# Autodesk Inventor assembly: MG996R_Servo_Motor_WithHorn
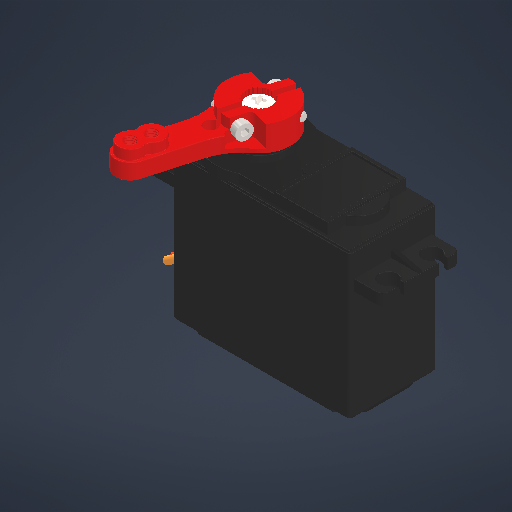
[picture p0: Inventor's stored thumbnail of the model, 512x512]
Saved by Autodesk Inventor 2025.2 (Build 292293000, 293)
## iProperties
Created: 2023-11-19
Part Number: MG996R_Servo_Motor_WithHorn
Document SubType Name: Assembly
Designer: Tiago
Sending System: SolidWorks 2022
Last Author: Ayman
Last Saved: 2023-12-26
Author: Tiago
## Documents named in this file (7)
- C:\Users\Tiago\Documents\Inventor\Exp. Braço v1\MG996R_Servo_Motor_WithHorn.iam
- C:\Users\Tiago\Documents\Inventor\Exp. Braço v1\MG996R Servo Motor\MG996R Servo Motor\MG996R Servo Motor\Case.ipt
- C:\Users\Tiago\Documents\Inventor\Exp. Braço v1\MG996R Servo Motor\MG996R Servo Motor\MG996R Servo Motor\Output Shaft.ipt
- C:\Users\Tiago\Documents\Inventor\Exp. Braço v1\MG996R Servo Motor\MG996R Servo Motor\MG996R Servo Motor\Rubber Wire Cable Sleeve.ipt
- C:\Users\Tiago\Documents\Inventor\Exp. Braço v1\MG996R Servo Motor\MG996R Servo Motor\MG996R Servo Motor\Pan Head Cross Screw M1.6.ipt
- C:\Users\Tiago\Documents\Inventor\Exp. Braço v1\MG996R Servo Motor\MG996R Servo Motor\MG996R Servo Motor\Pan Head Cross Screw M3.ipt
- C:\Users\Tiago\Documents\Inventor\Exp. Braço v1\SERVO ARM HORN 25T ALUMINIUM\SERVO ARM HORN WITH FASTENERS\SERVO ARM HORN WITH FASTENERS\SERVO ARM HORN WITH FASTENERS.iam
## Components (9 placed, 6 different names)
1. Case:1 — Flush:1, Mate:1, Insert:2, Insert:3, Insert:4, Insert:5, Mate:3
2. Output Shaft:1 — Flush:1, Mate:1, Mate:4
3. Rubber Wire Cable Sleeve:1
4. Pan Head Cross Screw M1.6:1 — Insert:3
5. Pan Head Cross Screw M1.6:2 — Insert:4
6. Pan Head Cross Screw M1.6:3 — Insert:5
7. Pan Head Cross Screw M1.6:4 — Insert:2
8. Pan Head Cross Screw M3:1 — Mate:2, Mate:4
9. SERVO ARM HORN WITH FASTENERS:1 [sub-assembly] — Mate:2, Mate:3
## Relationships (9: Mate 4, Insert 4, Flush 1)
- Flush:1 (-3.7 mm): Case:1 ↔ Output Shaft:1
- Mate:1: Case:1 ↔ Output Shaft:1
- Insert:2: Case:1 ↔ Pan Head Cross Screw M1.6:4
- Insert:3: Case:1 ↔ Pan Head Cross Screw M1.6:1
- Insert:4: Case:1 ↔ Pan Head Cross Screw M1.6:2
- Insert:5: Case:1 ↔ Pan Head Cross Screw M1.6:3
- Mate:2: Pan Head Cross Screw M3:1 ↔ SERVO ARM HORN WITH FASTENERS:1
- Mate:3 (0.5 mm): Case:1 ↔ SERVO ARM HORN WITH FASTENERS:1
- Mate:4: Output Shaft:1 ↔ Pan Head Cross Screw M3:1
